# Autodesk Inventor assembly: Tire
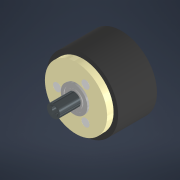
[picture p0: Inventor's stored thumbnail of the model, 180x180]
Saved by Autodesk Inventor 2022 (Build 260153000, 153)
## iProperties
Created: 2021-09-23
Part Number: Tire
Document SubType Name: Assembly
Designer: shiok
Mass: 6.37362 g
Surface Area: 59.289 cm^2
Volume: 3.61915 cm^3
Density: 1.76108 g/cm^3
Author: shiok
## Documents named in this file (7)
- C:\Users\shiok\Documents\GitHub\murakumo\inventor\Tire.iam
- C:\Users\shiok\Documents\GitHub\murakumo\inventor\wheel.ipt
- C:\Users\shiok\Documents\GitHub\murakumo\inventor\wheelcap.ipt
- C:\Users\shiok\Documents\GitHub\murakumo\inventor\Tire.ipt
- C:\Users\shiok\Documents\GitHub\murakumo\inventor\spergear.ipt
- C:\Users\shiok\Documents\GitHub\murakumo\inventor\FL674ZZ.ipt
- C:\Users\shiok\Documents\GitHub\murakumo\inventor\shaft.ipt
## Components (8 placed, 6 different names)
1. wheel:1 — 挿入:1, 挿入:2, メイト:1, 挿入:3, メイト:4, メイト:5
2. wheelcap:1 — 挿入:1, メイト:6, メイト:7
3. Tire:1 — 挿入:2
4. spergear:1 — メイト:1, 挿入:3, メイト:2, メイト:3
5. FL674ZZ:1 — メイト:2, メイト:3
6. FL674ZZ:2 — メイト:4, メイト:5
7. FL674ZZ:3 — メイト:6, メイト:7, フラッシュ:9, 挿入:4
8. shaft:1 — フラッシュ:9, 挿入:4
## Relationships (12: Mate 7, Insert 4, Flush 1)
- 挿入:1 [Insert]: wheel:1 ↔ wheelcap:1
- 挿入:2 [Insert]: wheel:1 ↔ Tire:1
- メイト:1 [Mate]: wheel:1 ↔ spergear:1
- 挿入:3 [Insert]: wheel:1 ↔ spergear:1
- メイト:2 [Mate]: spergear:1 ↔ FL674ZZ:1
- メイト:3 [Mate]: spergear:1 ↔ FL674ZZ:1
- メイト:4 [Mate]: wheel:1 ↔ FL674ZZ:2
- メイト:5 [Mate]: wheel:1 ↔ FL674ZZ:2
- メイト:6 [Mate]: wheelcap:1 ↔ FL674ZZ:3
- メイト:7 [Mate]: wheelcap:1 ↔ FL674ZZ:3
- フラッシュ:9 [Flush]: FL674ZZ:3 ↔ shaft:1
- 挿入:4 [Insert]: FL674ZZ:3 ↔ shaft:1
